# Autodesk Inventor assembly: Face Mask Assembly
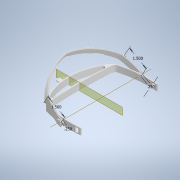
[picture p0: Inventor's stored thumbnail of the model, 180x180]
Saved by Autodesk Inventor 2020 (Build 240168000, 168)
## iProperties
Created: 2020-04-12
Part Number: Face Mask Assembly
Document SubType Name: Assembly
Designer: maple
Author: maple
## Documents named in this file (3)
- C:\Users\maple\Desktop\FaceShield_Assembly.iam
- C:\Users\maple\Desktop\FaceShield_Part2.ipt
- C:\Users\maple\Desktop\FaceShield_Part1.ipt
## Components (2 placed, 2 different names)
1. FaceShield_Part2:1 — Mate:1, Flush:1
2. FaceShield_Part1:1 — Mate:1, Flush:1
## Relationships (2: Mate 1, Flush 1)
- Mate:1: FaceShield_Part2:1 ↔ FaceShield_Part1:1
- Flush:1: FaceShield_Part2:1 ↔ FaceShield_Part1:1
